# Autodesk Inventor assembly: MotorAssembly
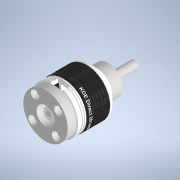
[picture p0: Inventor's stored thumbnail of the model, 180x180]
Saved by Autodesk Inventor 2022 (Build 260153000, 153)
## iProperties
Created: 2022-02-05
Part Number: MotorAssembly
Document SubType Name: Assembly
Designer: ultra
Author: ultra
## Documents named in this file (4)
- C:\Users\ultra\Desktop\RAS Aerial\MotorAssembly.iam
- C:\Users\ultra\Desktop\RAS Aerial\KDE2814XF-SERIES.iam
- C:\Users\ultra\Desktop\RAS Aerial\MotorAdaptor.ipt
- C:\Users\ultra\Desktop\RAS Aerial\MotorMount.ipt
## Components (3 placed, 3 different names)
1. KDE2814XF-SERIES:1 [sub-assembly] — Insert:1, Insert:2
2. MotorAdaptor:1 — Insert:1
3. MotorMount:1 — Insert:2
## Relationships (2: Insert 2)
- Insert:1: KDE2814XF-SERIES:1 ↔ MotorAdaptor:1
- Insert:2: KDE2814XF-SERIES:1 ↔ MotorMount:1
